# Autodesk Inventor assembly: Vòng Bi
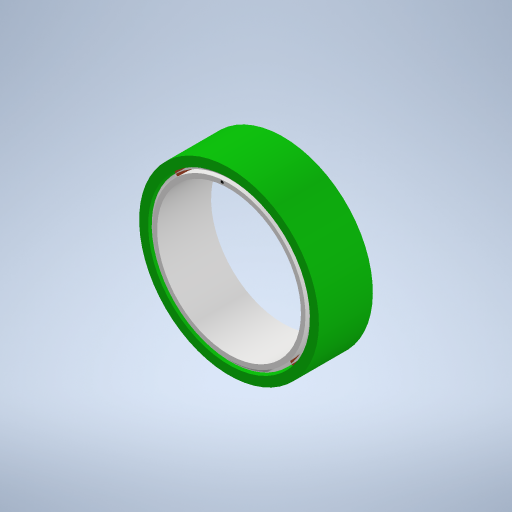
[picture p0: Inventor's stored thumbnail of the model, 512x512]
Saved by Autodesk Inventor 2023 (Build 270158000, 158)
## iProperties
Created: 2023-10-09
Part Number: Vòng Bi
Document SubType Name: Assembly
Designer: huy20
Author: huy20
## Documents named in this file (5)
- C:\Users\huy20\OneDrive\Máy tính\Inventor\TK Cơ cấu cơ khi\Chi tiết\Máy Nén Khí\Vòng Bi.iam
- C:\Users\huy20\OneDrive\Máy tính\Inventor\TK Cơ cấu cơ khi\Chi tiết\Máy Nén Khí\Vòng Bi\Bi.ipt
- C:\Users\huy20\OneDrive\Máy tính\Inventor\TK Cơ cấu cơ khi\Chi tiết\Máy Nén Khí\Vòng Bi\In1.ipt
- C:\Users\huy20\OneDrive\Máy tính\Inventor\TK Cơ cấu cơ khi\Chi tiết\Máy Nén Khí\Vòng Bi\Lock.ipt
- C:\Users\huy20\OneDrive\Máy tính\Inventor\TK Cơ cấu cơ khi\Chi tiết\Máy Nén Khí\Vòng Bi\Out.ipt
## Components (15 placed, 4 different names)
1. Bi:1 — Insert:12
2. In1:1 — Mate:1, Mate:2, Angle:1, Mate:3, Flush:1, Mate:4
3. Lock:1 — Insert:1, Insert:2, Insert:3, Insert:4, Insert:5, Insert:6, Insert:7, Insert:8, Insert:9, Insert:10, Insert:11, Insert:12, Mate:1, Mate:2, Angle:1
4. Out:1 — Mate:3, Flush:1
5. Bi:2 — Insert:9
6. Bi:3 — Insert:3
7. Bi:4 — Insert:5
8. Bi:5 — Insert:11
9. Bi:6 — Insert:8
10. Bi:7 — Insert:7
11. Bi:8 — Insert:6
12. Bi:9 — Insert:4
13. Bi:10 — Insert:1
14. Bi:11 — Insert:2
15. Bi:12 — Insert:10
## Relationships (18: Insert 12, Mate 4, Angle 1, Flush 1)
- Insert:1: Lock:1 ↔ Bi:10
- Insert:2: Lock:1 ↔ Bi:11
- Insert:3: Lock:1 ↔ Bi:3
- Insert:4: Lock:1 ↔ Bi:9
- Insert:5: Lock:1 ↔ Bi:4
- Insert:6: Lock:1 ↔ Bi:8
- Insert:7: Lock:1 ↔ Bi:7
- Insert:8: Lock:1 ↔ Bi:6
- Insert:9: Lock:1 ↔ Bi:2
- Insert:10: Lock:1 ↔ Bi:12
- Insert:11: Lock:1 ↔ Bi:5
- Insert:12: Bi:1 ↔ Lock:1
- Mate:1: In1:1 ↔ Lock:1
- Mate:2: In1:1 ↔ Lock:1
- Angle:1 (462 deg): In1:1 ↔ Lock:1
- Mate:3: In1:1 ↔ Out:1
- Flush:1: In1:1 ↔ Out:1
- Mate:4: In1:1
